# Autodesk Inventor assembly: 上半身
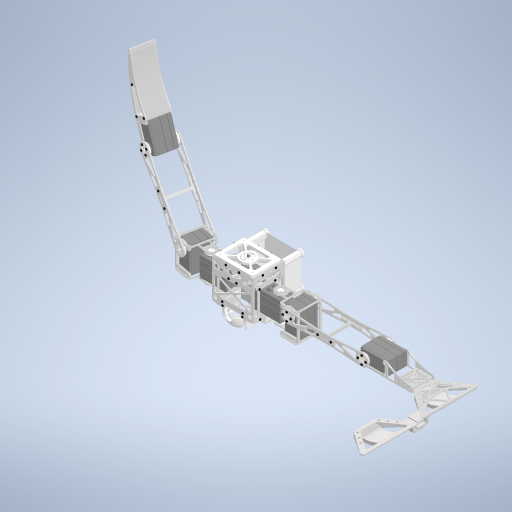
[picture p0: Inventor's stored thumbnail of the model, 512x512]
Saved by Autodesk Inventor 2024 (Build 280153000, 153)
## iProperties
Created: 2023-03-27
Part Number: 上半身
Document SubType Name: Assembly
Designer: right
Mass: 520.221 g
Surface Area: 2039.62 cm^2
Volume: 304.319 cm^3
Density: 1.70946 g/cm^3
Author: right
## Documents named in this file (22)
- C:\Users\right\OneDrive\ドキュメント\Inventor\V2二足Light＿仮\上半身.iam
- C:\Users\right\OneDrive\ドキュメント\Inventor\V2二足Light＿仮\上半身↓.ipt
- C:\Users\right\OneDrive\ドキュメント\Inventor\V2二足Light＿仮\02157_SmallDiameterHornB.ipt
- C:\Users\right\OneDrive\ドキュメント\Inventor\V2二足Light＿仮\back.ipt
- C:\Users\right\OneDrive\ドキュメント\Inventor\V2二足Light＿仮\waki.ipt
- C:\Users\right\OneDrive\ドキュメント\Inventor\V2二足Light＿仮\mune.ipt
- C:\Users\right\OneDrive\ドキュメント\Inventor\V2二足Light＿仮\ude.iam
- C:\Users\right\OneDrive\ドキュメント\Inventor\V2二足Light＿仮\waki_2_MIR.ipt
- C:\Users\right\OneDrive\ドキュメント\EAGLE\projects\V2_2soku v0.iam
- C:\Users\right\OneDrive\ドキュメント\Inventor\V2二足Light＿仮\Lzi.ipt
- D:\inventor\二足歩行ロボット\jusin.ipt
- C:\Users\right\OneDrive\ドキュメント\Inventor\V2二足Light＿仮\face.ipt
- C:\Users\right\OneDrive\ドキュメント\Inventor\V2二足Light＿仮\batcase.ipt
- C:\Users\right\OneDrive\ドキュメント\Inventor\V2二足Light＿仮\M2小ねじ.ipt
- C:\Users\right\OneDrive\ドキュメント\Inventor\V2二足Light＿仮\M2小ねじ1.ipt
- C:\Users\right\OneDrive\ドキュメント\Inventor\V2二足Light＿仮\M3中ねじ.ipt
- C:\Users\right\OneDrive\ドキュメント\Inventor\V2二足Light＿仮\ude_MIR.iam
- C:\Users\right\OneDrive\ドキュメント\Inventor\V2二足Light＿仮\kshi_zikuuke.ipt
- C:\Users\right\OneDrive\ドキュメント\Inventor\V2二足Light＿仮\基板保護.ipt
- C:\Users\right\OneDrive\ドキュメント\Inventor\V2二足Light＿仮\基板保護↑.ipt
- C:\Users\right\OneDrive\ドキュメント\Inventor\V2二足Light＿仮\batcace_under.ipt
- C:\Users\right\OneDrive\ドキュメント\Inventor\V2二足Light＿仮\bat.ipt
## Components (54 placed, 21 different names)
1. 上半身↓:1 — 挿入:1, 挿入:2, 挿入:3, 挿入:4, 挿入:5, 挿入:8, 挿入:9, 挿入:26, 挿入:27, 挿入:32, 挿入:38, 挿入:63, 挿入:64, 挿入:65, 挿入:66, フラッシュ:4, メイト:1
2. 02157_SmallDiameterHornB:1 — 挿入:1, 挿入:2, 挿入:3, 挿入:79
3. back:1 — 挿入:4, 挿入:5, 挿入:22, 挿入:23, フラッシュ:3, 挿入:59, 挿入:60, 挿入:61, 挿入:62, 挿入:86, 挿入:87, 挿入:88, 挿入:89, メイト:2
4. waki:2 — 挿入:8, 挿入:9, 挿入:35, 挿入:82, 挿入:83
5. ude:1 [sub-assembly] — 挿入:33, 挿入:67, 挿入:68, 挿入:69
6. V2_2soku v0:1 [sub-assembly] — 挿入:22, 挿入:23
7. mune:1 — 挿入:26, 挿入:27, 挿入:36, 挿入:41, 挿入:42, 挿入:47, 挿入:48, 挿入:49, 挿入:50, 挿入:51, 挿入:52, 挿入:80, 挿入:81
8. waki:3 — 挿入:32, 挿入:38, 挿入:53, 挿入:54, 挿入:55, 挿入:56, 挿入:57, 挿入:58
9. Lzi:1 — フラッシュ:3, 挿入:43, 挿入:44, 挿入:45, 挿入:46, 挿入:75, 挿入:76, メイト:3
10. waki_2_MIR:1 — 挿入:33, 挿入:35, 挿入:36
11. jusin:1 — 挿入:41, 挿入:42
12. face:1 — 挿入:43, 挿入:44
13. batcase:1 — 挿入:45, 挿入:46, フラッシュ:5
14. M2小ねじ:1 — 挿入:47
15. M2小ねじ:2 — 挿入:48
16. M2小ねじ:3 — 挿入:49
17. M2小ねじ:4 — 挿入:50
18. M2小ねじ:5 — 挿入:52
19. M2小ねじ:6 — 挿入:51
20. M2小ねじ:7 — 挿入:54
21. M2小ねじ:8 — 挿入:53
22. M2小ねじ:9 — 挿入:56
23. M2小ねじ:10 — 挿入:55
24. M2小ねじ:11 — 挿入:57
25. M2小ねじ:12 — 挿入:58
26. M2小ねじ1:1
27. M2小ねじ1:2
28. M2小ねじ1:3
29. M2小ねじ1:4
30. M2小ねじ1:5 — 挿入:82
31. M2小ねじ1:6 — 挿入:83
32. M2小ねじ:13 — 挿入:60
33. M2小ねじ:14 — 挿入:59
34. M2小ねじ:15 — 挿入:61
35. M2小ねじ:16 — 挿入:62
36. M2小ねじ:17 — 挿入:64
37. M2小ねじ:18 — 挿入:63
38. M2小ねじ:19 — 挿入:66
39. M2小ねじ:20 — 挿入:65
40. M2小ねじ:26 — 挿入:69
41. M2小ねじ:27 — 挿入:68
42. M2小ねじ:28 — 挿入:67
43. M2小ねじ:29 — 挿入:75
44. M2小ねじ:30 — 挿入:76
45. M3中ねじ:1 — 挿入:79
46. M2小ねじ:31 — 挿入:80
47. M2小ねじ:32 — 挿入:81
48. ude_MIR:1 [sub-assembly]
49. kshi_zikuuke:1 — フラッシュ:4
50. 基板保護:1 — 挿入:88, 挿入:89, 挿入:91
51. 基板保護:2 — 挿入:86, 挿入:87, 挿入:90
52. 基板保護↑:1 — 挿入:90, 挿入:91
53. batcace_under:1 — フラッシュ:5
54. bat:1 — メイト:1, メイト:2, メイト:3
## Relationships (64: Insert 58, Flush 3, Mate 3)
- 挿入:1 [Insert]: 上半身↓:1 ↔ 02157_SmallDiameterHornB:1
- 挿入:2 [Insert]: 上半身↓:1 ↔ 02157_SmallDiameterHornB:1
- 挿入:3 [Insert]: 上半身↓:1 ↔ 02157_SmallDiameterHornB:1
- 挿入:4 [Insert]: 上半身↓:1 ↔ back:1
- 挿入:5 [Insert]: 上半身↓:1 ↔ back:1
- 挿入:8 [Insert]: 上半身↓:1 ↔ waki:2
- 挿入:9 [Insert]: 上半身↓:1 ↔ waki:2
- 挿入:22 [Insert] (2 mm): back:1 ↔ V2_2soku v0:1
- 挿入:23 [Insert] (2 mm): back:1 ↔ V2_2soku v0:1
- 挿入:26 [Insert]: 上半身↓:1 ↔ mune:1
- 挿入:27 [Insert]: 上半身↓:1 ↔ mune:1
- 挿入:32 [Insert]: 上半身↓:1 ↔ waki:3
- フラッシュ:3 [Flush]: back:1 ↔ Lzi:1
- 挿入:33 [Insert]: ude:1 ↔ waki_2_MIR:1
- 挿入:35 [Insert]: waki:2 ↔ waki_2_MIR:1
- 挿入:36 [Insert]: mune:1 ↔ waki_2_MIR:1
- 挿入:38 [Insert]: 上半身↓:1 ↔ waki:3
- 挿入:41 [Insert]: mune:1 ↔ jusin:1
- 挿入:42 [Insert]: mune:1 ↔ jusin:1
- 挿入:43 [Insert]: Lzi:1 ↔ face:1
- 挿入:44 [Insert]: Lzi:1 ↔ face:1
- 挿入:45 [Insert] (12 mm): Lzi:1 ↔ batcase:1
- 挿入:46 [Insert] (12 mm): Lzi:1 ↔ batcase:1
- 挿入:47 [Insert]: mune:1 ↔ M2小ねじ:1
- 挿入:48 [Insert]: mune:1 ↔ M2小ねじ:2
- 挿入:49 [Insert]: mune:1 ↔ M2小ねじ:3
- 挿入:50 [Insert]: mune:1 ↔ M2小ねじ:4
- 挿入:51 [Insert]: mune:1 ↔ M2小ねじ:6
- 挿入:52 [Insert]: mune:1 ↔ M2小ねじ:5
- 挿入:53 [Insert]: waki:3 ↔ M2小ねじ:8
- 挿入:54 [Insert]: waki:3 ↔ M2小ねじ:7
- 挿入:55 [Insert]: waki:3 ↔ M2小ねじ:10
- 挿入:56 [Insert]: waki:3 ↔ M2小ねじ:9
- 挿入:57 [Insert]: waki:3 ↔ M2小ねじ:11
- 挿入:58 [Insert]: waki:3 ↔ M2小ねじ:12
- 挿入:59 [Insert]: back:1 ↔ M2小ねじ:14
- 挿入:60 [Insert]: back:1 ↔ M2小ねじ:13
- 挿入:61 [Insert]: back:1 ↔ M2小ねじ:15
- 挿入:62 [Insert]: back:1 ↔ M2小ねじ:16
- 挿入:63 [Insert]: 上半身↓:1 ↔ M2小ねじ:18
- 挿入:64 [Insert]: 上半身↓:1 ↔ M2小ねじ:17
- 挿入:65 [Insert]: 上半身↓:1 ↔ M2小ねじ:20
- 挿入:66 [Insert]: 上半身↓:1 ↔ M2小ねじ:19
- 挿入:67 [Insert]: ude:1 ↔ M2小ねじ:28
- 挿入:68 [Insert]: ude:1 ↔ M2小ねじ:27
- 挿入:69 [Insert]: ude:1 ↔ M2小ねじ:26
- 挿入:75 [Insert]: Lzi:1 ↔ M2小ねじ:29
- 挿入:76 [Insert]: Lzi:1 ↔ M2小ねじ:30
- 挿入:79 [Insert]: 02157_SmallDiameterHornB:1 ↔ M3中ねじ:1
- 挿入:80 [Insert]: mune:1 ↔ M2小ねじ:31
- 挿入:81 [Insert]: mune:1 ↔ M2小ねじ:32
- 挿入:82 [Insert]: waki:2 ↔ M2小ねじ1:5
- 挿入:83 [Insert]: waki:2 ↔ M2小ねじ1:6
- フラッシュ:4 [Flush]: 上半身↓:1 ↔ kshi_zikuuke:1
- 挿入:86 [Insert]: back:1 ↔ 基板保護:2
- 挿入:87 [Insert]: back:1 ↔ 基板保護:2
- 挿入:88 [Insert]: back:1 ↔ 基板保護:1
- 挿入:89 [Insert]: back:1 ↔ 基板保護:1
- 挿入:90 [Insert]: 基板保護:2 ↔ 基板保護↑:1
- 挿入:91 [Insert]: 基板保護:1 ↔ 基板保護↑:1
- フラッシュ:5 [Flush]: batcase:1 ↔ batcace_under:1
- メイト:1 [Mate]: 上半身↓:1 ↔ bat:1
- メイト:2 [Mate]: back:1 ↔ bat:1
- メイト:3 [Mate]: Lzi:1 ↔ bat:1
